# Autodesk Inventor assembly: Testing assembly
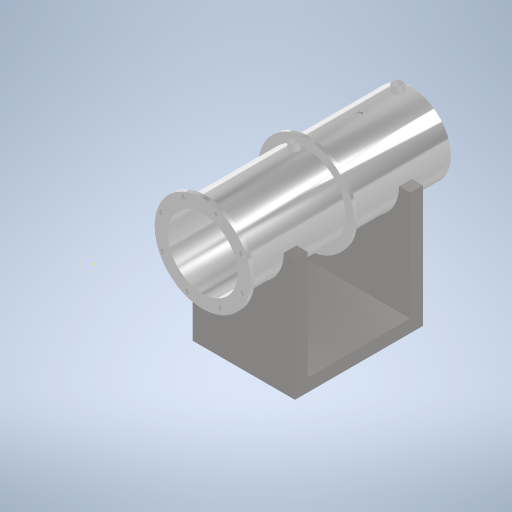
[picture p0: Inventor's stored thumbnail of the model, 512x512]
Saved by Autodesk Inventor 2023 (Build 270158000, 158)
## iProperties
Created: 2022-09-29
Part Number: Testing assembly
Document SubType Name: Assembly
Designer: station
Author: station
## Documents named in this file (3)
- C:\Users\station\Documents\Project\Liquid-engine-cooling-system\design files\ethanol engine 6\Aluminium engine v2\Testing assembly.iam
- C:\Users\station\Documents\Project\Liquid-engine-cooling-system\design files\ethanol engine 6\Aluminium engine v2\support assembly.iam
- C:\Users\station\Documents\Project\Liquid-engine-cooling-system\design files\ethanol engine 6\Aluminium engine v2\aluminium engine v2.iam
## Components (2 placed, 2 different names)
1. support assembly:1 [sub-assembly] — Mate:1
2. aluminium engine v2:1 [sub-assembly] — Mate:1
## Relationships (1: Mate 1)
- Mate:1: support assembly:1 ↔ aluminium engine v2:1
